# Autodesk Inventor assembly: Cópia
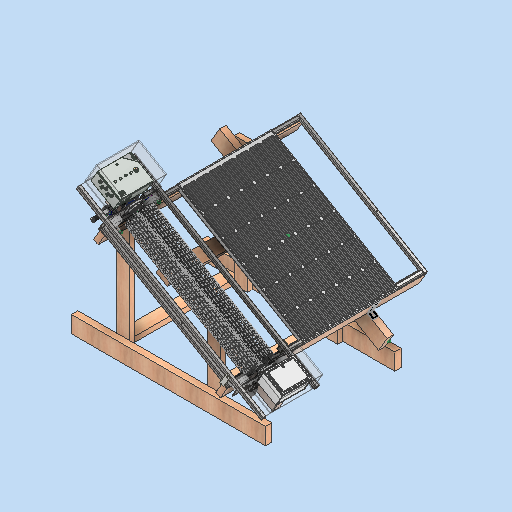
[picture p0: Inventor's stored thumbnail of the model, 512x512]
Saved by Autodesk Inventor 2026.2 (Build 302298010, 298A)
## iProperties
Created: 2019-12-15
Part Number: Cópia
Document SubType Name: Assembly
Designer: Rubens
Sending System: SolidWorks 2021
Last Author: Mohsen
Last Saved: 2022-08-25
Author: Rubens
## Documents named in this file (21)
- C:\Users\Rubens\Downloads\Estrutura de madeira\TCC 1204\TCC 1204\TCC 1004\TCC 3103\TCC 3003\TCC 2903\TCC1803\TCC 1703\Projeto TCC\Main_Solar_Structure\Montagem com painel menor.iam
- C:\Users\Rubens\Downloads\Estrutura de madeira\TCC 1204\TCC 1204\TCC 1004\TCC 3103\TCC 3003\TCC 2903\TCC1803\TCC 1703\Projeto TCC\Main_Solar_Structure\Small_Column.ipt
- C:\Users\Rubens\Downloads\Estrutura de madeira\TCC 1204\TCC 1204\TCC 1004\TCC 3103\TCC 3003\TCC 2903\TCC1803\TCC 1703\Projeto TCC\Main_Solar_Structure\Large_Column.ipt
- C:\Users\Rubens\Downloads\Estrutura de madeira\TCC 1204\TCC 1204\TCC 1004\TCC 3103\TCC 3003\TCC 2903\TCC1803\TCC 1703\Projeto TCC\Main_Solar_Structure\Bottom_Beam.ipt
- C:\Users\Rubens\Downloads\Estrutura de madeira\TCC 1204\TCC 1204\TCC 1004\TCC 3103\TCC 3003\TCC 2903\TCC1803\TCC 1703\Projeto TCC\Main_Solar_Structure\Beam_Support.ipt
- C:\Users\Rubens\Downloads\Estrutura de madeira\TCC 1204\TCC 1204\TCC 1004\TCC 3103\TCC 3003\TCC 2903\TCC1803\TCC 1703\Projeto TCC\Main_Solar_Structure\M10_Screw&Nut.iam
- C:\Users\Rubens\Downloads\Estrutura de madeira\TCC 1204\TCC 1204\TCC 1004\TCC 3103\TCC 3003\TCC 2903\TCC1803\TCC 1703\Projeto TCC\Main_Solar_Structure\Top_Beam_2780.ipt
- C:\Users\Rubens\Downloads\Estrutura de madeira\TCC 1204\TCC 1204\TCC 1004\TCC 3103\TCC 3003\TCC 2903\TCC1803\TCC 1703\Projeto TCC\Main_Solar_Structure\Perfil tubo - 30x30x3.ipt
- C:\Users\Rubens\Downloads\Estrutura de madeira\TCC 1204\TCC 1204\TCC 1004\TCC 3103\TCC 3003\TCC 2903\TCC1803\TCC 1703\Projeto TCC\Main_Solar_Structure\tubo 30 x 30 x 3  - 500.ipt
- C:\Users\Rubens\Downloads\Estrutura de madeira\TCC 1204\TCC 1204\TCC 1004\TCC 3103\TCC 3003\TCC 2903\TCC1803\TCC 1703\Projeto TCC\Projeto Limpador\PV ST SOLAR.ipt
- C:\Users\Rubens\Downloads\Estrutura de madeira\TCC 1204\TCC 1204\TCC 1004\TCC 3103\TCC 3003\TCC 2903\TCC1803\TCC 1703\Projeto TCC\Main_Solar_Structure\Small_Column_MIR3.ipt
- C:\Users\Rubens\Downloads\Estrutura de madeira\TCC 1204\TCC 1204\TCC 1004\TCC 3103\TCC 3003\TCC 2903\TCC1803\TCC 1703\Projeto TCC\Main_Solar_Structure\Bottom_Beam_MIR3.ipt
- C:\Users\Rubens\Downloads\Estrutura de madeira\TCC 1204\TCC 1204\TCC 1004\TCC 3103\TCC 3003\TCC 2903\TCC1803\TCC 1703\Projeto TCC\Main_Solar_Structure\Beam_Support_MIR2.ipt
- C:\Users\Rubens\Downloads\Estrutura de madeira\TCC 1204\TCC 1204\TCC 1004\TCC 3103\TCC 3003\TCC 2903\TCC1803\TCC 1703\Projeto TCC\Main_Solar_Structure\M10_Screw&Nut_MIR2.iam
- C:\Users\Rubens\Downloads\Estrutura de madeira\TCC 1204\TCC 1204\TCC 1004\TCC 3103\TCC 3003\TCC 2903\TCC1803\TCC 1703\Projeto TCC\Main_Solar_Structure\Large_Column_MIR4.ipt
- C:\Users\Rubens\Downloads\Estrutura de madeira\TCC 1204\TCC 1204\TCC 1004\TCC 3103\TCC 3003\TCC 2903\TCC1803\TCC 1703\Projeto TCC\Main_Solar_Structure\tubo extensão menor.ipt
- C:\Users\Rubens\Downloads\Estrutura de madeira\TCC 1204\TCC 1204\TCC 1004\TCC 3103\TCC 3003\TCC 2903\TCC1803\TCC 1703\Projeto TCC\Main_Solar_Structure\Madeira de sustentação-950.ipt
- C:\Users\Rubens\Downloads\Estrutura de madeira\TCC 1204\TCC 1204\TCC 1004\TCC 3103\TCC 3003\TCC 2903\TCC1803\TCC 1703\Projeto TCC\Main_Solar_Structure\Madeira de sustentação superior 870.ipt
- C:\Users\Rubens\Downloads\TCC 1204\TCC 1004\TCC 3103\TCC 3003\TCC 2903\TCC1803\TCC 1703\Projeto TCC\Projeto Limpador\MontagemREVXX.iam
- C:\Users\Rubens\Downloads\hc-sr04-ultrasonic-sensor-12.snapshot.1\Ultrasonic sensor\Ultrasonic sensor\Ultrasonic sensor.iam
- C:\Users\Rubens\Desktop\GIT TCC\mecanica\Chapa para sensor ultrassônico.ipt
## Components (45 placed, 20 different names)
1. Small_Column:1 — Flush:6, Mate:67, Flush:74, Mate:148
2. Bottom_Beam:1 — Mate:3, Mate:5, Mate:20, Mate:21, Mate:66, Angle:1, Mate:113, Mate:128, Flush:57, Flush:67, Mate:146, Flush:76
3. Beam_Support:3 — Mate:3, Mate:5, Mate:23
4. M10_Screw&Nut:2 [sub-assembly]
5. M10_Screw&Nut:7 [sub-assembly]
6. M10_Screw&Nut:8 [sub-assembly]
7. M10_Screw&Nut:9 [sub-assembly]
8. M10_Screw&Nut:90 [sub-assembly]
9. M10_Screw&Nut:91 [sub-assembly]
10. Top_Beam_2780:1 — Mate:21, Flush:7, Flush:45, Mate:112, Mate:129, Flush:59, Flush:67, Flush:75, Mate:161, Flush:90, Mate:166
11. Top_Beam_2780:2 — Mate:20, Mate:23, Flush:7, Mate:107, Flush:94, Flush:95
12. Large_Column:1 — Mate:66, Mate:67, Mate:144, Flush:72, Mate:149
13. M10_Screw&Nut:92 [sub-assembly]
14. M10_Screw&Nut:93 [sub-assembly]
15. M10_Screw&Nut:94 [sub-assembly]
16. M10_Screw&Nut:96 [sub-assembly]
17. PV ST SOLAR:1 — Mate:107, Flush:45, Tangent:1, Flush:78, Mate:162, Mate:165, Flush:93
18. Beam_Support:4 — Mate:112, Mate:113, Mate:128, Flush:57
19. Small_Column_MIR3:1 — Flush:55, Mate:121, Mate:145
20. Bottom_Beam_MIR3:1 — Mate:118, Mate:119, Mate:122, Angle:2, Mate:127, Flush:58, Flush:59
21. Beam_Support_MIR2:1 — Mate:118, Mate:119
22. M10_Screw&Nut_MIR2:1 [sub-assembly]
23. M10_Screw&Nut_MIR2:2 [sub-assembly]
24. M10_Screw&Nut_MIR2:3 [sub-assembly]
25. M10_Screw&Nut_MIR2:4 [sub-assembly]
26. Large_Column_MIR4:1 — Mate:121, Mate:122, Flush:73, Mate:151
27. M10_Screw&Nut_MIR2:5 [sub-assembly]
28. M10_Screw&Nut_MIR2:6 [sub-assembly]
29. M10_Screw&Nut_MIR2:7 [sub-assembly]
30. Beam_Support_MIR2:2 — Mate:127, Mate:129, Flush:58
31. Bottom_Beam:2 — Mate:144, Flush:72, Flush:74, Mate:147, Flush:77
32. Bottom_Beam:3 — Mate:145, Flush:73, Mate:150
33. Madeira de sustentação-950:1 — Mate:149, Mate:150, Mate:151
34. Madeira de sustentação-950:2 — Mate:147, Flush:77, Mate:148
35. Madeira de sustentação superior 870:1 — Mate:146, Flush:75, Flush:76
36. MontagemREVXX:1 [sub-assembly] — Tangent:1, Flush:78, Mate:154, Flush:80, Flush:81, Mate:155, Flush:82, Flush:83
37. Ultrasonic sensor:2 [sub-assembly]
38. Chapa para sensor ultrassônico:2 — Mate:154, Flush:80, Flush:81
39. Chapa para sensor ultrassônico:3 — Mate:155, Flush:82, Flush:83
40. tubo 30 x 30 x 3  - 500:6 — Mate:163, Flush:91, Mate:165, Mate:166, Flush:93
41. Perfil tubo - 30x30x3:8 — Mate:158, Mate:159, Flush:87, Mate:160, Flush:88
42. tubo extensão menor:3 — Mate:158, Mate:159, Flush:87, Flush:95
43. tubo extensão menor:5 — Mate:160, Flush:88, Mate:161, Flush:90, Mate:162
44. Perfil tubo - 30x30x3:9 — Mate:163, Flush:91, Mate:164, Flush:92, Flush:94
45. tubo 30 x 30 x 3  - 500:8 — Mate:164, Flush:92
## Relationships (67: Mate 36, Flush 28, Angle 2, Tangent 1)
- Mate:3: Bottom_Beam:1 ↔ Beam_Support:3
- Mate:5: Bottom_Beam:1 ↔ Beam_Support:3
- Flush:6 (300 mm): Small_Column:1
- Mate:20: Bottom_Beam:1 ↔ Top_Beam_2780:2
- Mate:21: Bottom_Beam:1 ↔ Top_Beam_2780:1
- Mate:23: Beam_Support:3 ↔ Top_Beam_2780:2
- Flush:7: Top_Beam_2780:1 ↔ Top_Beam_2780:2
- Mate:66: Bottom_Beam:1 ↔ Large_Column:1
- Mate:67 (600 mm): Small_Column:1 ↔ Large_Column:1
- Angle:1 (0 deg): Bottom_Beam:1
- Flush:16 (-450 mm)
- Mate:107: Top_Beam_2780:2 ↔ PV ST SOLAR:1
- Flush:45: Top_Beam_2780:1 ↔ PV ST SOLAR:1
- Mate:112: Top_Beam_2780:1 ↔ Beam_Support:4
- Mate:113: Bottom_Beam:1 ↔ Beam_Support:4
- Mate:118: Bottom_Beam_MIR3:1 ↔ Beam_Support_MIR2:1
- Mate:119: Bottom_Beam_MIR3:1 ↔ Beam_Support_MIR2:1
- Flush:55 (300 mm): Small_Column_MIR3:1
- Mate:121 (600 mm): Small_Column_MIR3:1 ↔ Large_Column_MIR4:1
- Mate:122: Bottom_Beam_MIR3:1 ↔ Large_Column_MIR4:1
- Angle:2 (0 deg): Bottom_Beam_MIR3:1
- Mate:127: Bottom_Beam_MIR3:1 ↔ Beam_Support_MIR2:2
- Mate:128: Bottom_Beam:1 ↔ Beam_Support:4
- Flush:57: Bottom_Beam:1 ↔ Beam_Support:4
- Mate:129: Top_Beam_2780:1 ↔ Beam_Support_MIR2:2
- Flush:58: Bottom_Beam_MIR3:1 ↔ Beam_Support_MIR2:2
- Flush:59 (180 mm): Top_Beam_2780:1 ↔ Bottom_Beam_MIR3:1
- Flush:67 (-315 mm): Bottom_Beam:1 ↔ Top_Beam_2780:1
- Mate:144: Large_Column:1 ↔ Bottom_Beam:2
- Flush:72 (-300 mm): Large_Column:1 ↔ Bottom_Beam:2
- Mate:145: Small_Column_MIR3:1 ↔ Bottom_Beam:3
- Flush:73 (-300 mm): Large_Column_MIR4:1 ↔ Bottom_Beam:3
- Flush:74: Small_Column:1 ↔ Bottom_Beam:2
- Mate:146: Bottom_Beam:1 ↔ Madeira de sustentação superior 870:1
- Flush:75 (-800 mm): Top_Beam_2780:1 ↔ Madeira de sustentação superior 870:1
- Flush:76: Bottom_Beam:1 ↔ Madeira de sustentação superior 870:1
- Mate:147: Bottom_Beam:2 ↔ Madeira de sustentação-950:2
- Flush:77: Bottom_Beam:2 ↔ Madeira de sustentação-950:2
- Mate:148: Small_Column:1 ↔ Madeira de sustentação-950:2
- Mate:149: Large_Column:1 ↔ Madeira de sustentação-950:1
- Mate:150: Bottom_Beam:3 ↔ Madeira de sustentação-950:1
- Mate:151: Large_Column_MIR4:1 ↔ Madeira de sustentação-950:1
- Tangent:1: PV ST SOLAR:1 ↔ MontagemREVXX:1
- Flush:78: PV ST SOLAR:1 ↔ MontagemREVXX:1
- Mate:154: MontagemREVXX:1 ↔ Chapa para sensor ultrassônico:2
- Flush:80: MontagemREVXX:1 ↔ Chapa para sensor ultrassônico:2
- Flush:81 (290 mm): MontagemREVXX:1 ↔ Chapa para sensor ultrassônico:2
- Mate:155: MontagemREVXX:1 ↔ Chapa para sensor ultrassônico:3
- Flush:82 (295 mm): MontagemREVXX:1 ↔ Chapa para sensor ultrassônico:3
- Flush:83: MontagemREVXX:1 ↔ Chapa para sensor ultrassônico:3
- Mate:158: Perfil tubo - 30x30x3:8 ↔ tubo extensão menor:3
- Mate:159: Perfil tubo - 30x30x3:8 ↔ tubo extensão menor:3
- Flush:87: Perfil tubo - 30x30x3:8 ↔ tubo extensão menor:3
- Mate:160: Perfil tubo - 30x30x3:8 ↔ tubo extensão menor:5
- Flush:88: Perfil tubo - 30x30x3:8 ↔ tubo extensão menor:5
- Mate:161: Top_Beam_2780:1 ↔ tubo extensão menor:5
- Flush:90: Top_Beam_2780:1 ↔ tubo extensão menor:5
- Mate:162: PV ST SOLAR:1 ↔ tubo extensão menor:5
- Mate:163: tubo 30 x 30 x 3  - 500:6 ↔ Perfil tubo - 30x30x3:9
- Flush:91: tubo 30 x 30 x 3  - 500:6 ↔ Perfil tubo - 30x30x3:9
- Mate:164: Perfil tubo - 30x30x3:9 ↔ tubo 30 x 30 x 3  - 500:8
- Flush:92: Perfil tubo - 30x30x3:9 ↔ tubo 30 x 30 x 3  - 500:8
- Mate:165: PV ST SOLAR:1 ↔ tubo 30 x 30 x 3  - 500:6
- Mate:166: Top_Beam_2780:1 ↔ tubo 30 x 30 x 3  - 500:6
- Flush:93: PV ST SOLAR:1 ↔ tubo 30 x 30 x 3  - 500:6
- Flush:94: Top_Beam_2780:2 ↔ Perfil tubo - 30x30x3:9
- Flush:95: Top_Beam_2780:2 ↔ tubo extensão menor:3
